# Autodesk Inventor assembly: CycloidalDrive2
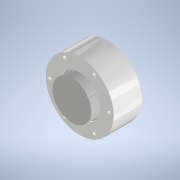
[picture p0: Inventor's stored thumbnail of the model, 180x180]
Saved by Autodesk Inventor 2022 (Build 260153000, 153)
## iProperties
Created: 2022-10-07
Part Number: CycloidalDrive2
Document SubType Name: Assembly
Designer: MicnedSQ
Author: MicnedSQ
## Documents named in this file (4)
- C:\Users\Micne\Desktop\RobotArmV1\RotatingBase\CycloidalDrive\CycloidalDrive2.iam
- C:\Users\Micne\Desktop\RobotArmV1\RotatingBase\CycloidalDrive\Bottom.ipt
- C:\Users\Micne\Desktop\RobotArmV1\RotatingBase\CycloidalDrive\OutputShaft.iam
- C:\Users\Micne\Desktop\RobotArmV1\RotatingBase\CycloidalDrive\CycloidalDisc.ipt
## Components (3 placed, 3 different names)
1. Bottom:1 — Obrotowe:1
2. OutputShaft:1 [sub-assembly] — Obrotowe:1, Rotational:2, Tangent:1, Tangent:2
3. CycloidalDisc:1 — Rotational:2, Tangent:1, Tangent:2
## Relationships (4: RevoluteJoint 2, Tangent 2)
- Obrotowe:1 [RevoluteJoint]: Bottom:1 ↔ OutputShaft:1
- Rotational:2 [RevoluteJoint]: OutputShaft:1 ↔ CycloidalDisc:1
- Tangent:1: OutputShaft:1 ↔ CycloidalDisc:1
- Tangent:2: OutputShaft:1 ↔ CycloidalDisc:1
